# Autodesk Inventor assembly: Assembly Estrutura
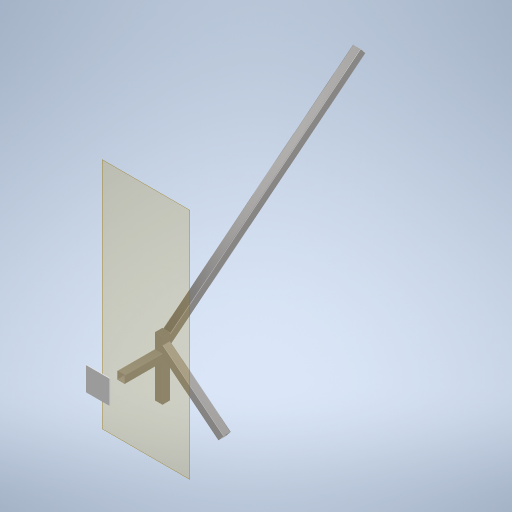
[picture p0: Inventor's stored thumbnail of the model, 512x512]
Saved by Autodesk Inventor 2024 (Build 280153000, 153)
## iProperties
Created: 2024-05-06
Part Number: Assembly Estrutura
Document SubType Name: Assembly
Designer: Pedro
Mass: 78864.6 g
Surface Area: 41238.5 cm^2
Volume: 10831.8 cm^3
Density: 7.28084 g/cm^3
Author: Pedro
_SolveAssemblyDoc: Frame Generator Solve Assembly
_Version: 25.0.0
## Documents named in this file (4)
- C:\Users\Pedro\Desktop\Autodesk Inbentor\Aula 11\Assembly Estrutura.iam
- C:\Users\Pedro\Desktop\Autodesk Inbentor\Aula 11\Estrutura.ipt
- C:\Users\Pedro\Desktop\Autodesk Inbentor\Aula 11\Assembly Estrutura\Frame\Frame 1714989157582.iam
- C:\Users\Pedro\Desktop\Autodesk Inbentor\Aula 11\Estrutura da Chapa.ipt
## Components (3 placed, 3 different names)
1. Estrutura:1
2. Frame 1714989157582:1 [sub-assembly] — Mate:1
3. Estrutura da Chapa:1 — Angle:1
## Relationships (2: Mate 1, Angle 1)
- Mate:1: Frame 1714989157582:1
- Angle:1 (0 deg): Estrutura da Chapa:1
